# Autodesk Inventor assembly: Lower Platform
Saved by Autodesk Inventor 2014 SP1 (Build 180222100, 222)
## iProperties
Created: 2013-12-29
Part Number: Lower Platform
Document SubType Name: Assembly
Designer: tom
Author: tom
## Documents named in this file (3)
- C:\Users\tom\Documents\GitHub\Delta_Robots\Delatabot - Small Model\Inventor\Deltabot - Small Model\Lower Platform.iam
- C:\Users\tom\Documents\GitHub\Delta_Robots\Delatabot - Small Model\Inventor\Deltabot - Small Model\Lower Platform.ipt
- C:\Users\tom\Documents\GitHub\Delta_Robots\Delatabot - Small Model\Inventor\Deltabot - Small Model\Lower Arm Bracket.ipt
## Components (4 placed, 2 different names)
1. Lower Base
2. Lower Arm Bracket:1
3. Lower Arm Bracket:2
4. Lower Arm Bracket:3
## Component patterns: (3 elements, first: Lower Arm Bracket:1)
## Relationships (3: Mate 3)
- [Mate]: Lower Base ↔ Lower Arm Bracket:1
- [Mate]: Lower Base ↔ Lower Arm Bracket:1
- [Mate]: Lower Base ↔ Lower Arm Bracket:1
